# Autodesk Inventor assembly: stresstestingassembly
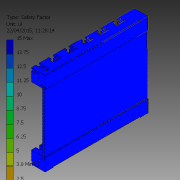
[picture p0: Inventor's stored thumbnail of the model, 180x180]
Saved by Autodesk Inventor 2015 (Build 190159000, 159)
## iProperties
Created: 2015-04-22
Part Number: stresstestingassembly
Document SubType Name: Assembly
Designer: Akovo_000
Author: Akovo_000
## Documents named in this file (9)
- C:\Users\Akovo_000\SkyDrive\3D printing\Enclosure Half-Open\stresstestingassembly.iam
- C:\Users\Akovo_000\SkyDrive\3D printing\Enclosure Half-Open\Pillar.ipt
- C:\Users\Akovo_000\SkyDrive\3D printing\Enclosure Half-Open\SidePanelNarrow.ipt
- C:\Users\Akovo_000\SkyDrive\3D printing\Enclosure Half-Open\stresstestingassembly\AIP\FEA\be9qf395s.fins
- C:\Users\Akovo_000\SkyDrive\3D printing\Enclosure Half-Open\stresstestingassembly\AIP\FEA\be9qf395s.fsat
- C:\Users\Akovo_000\SkyDrive\3D printing\Enclosure Half-Open\stresstestingassembly\AIP\FEA\be9qf396o.ftes
- C:\Users\Akovo_000\SkyDrive\3D printing\Enclosure Half-Open\stresstestingassembly\AIP\FEA\be9qf396o.fwiz
- C:\Users\Akovo_000\SkyDrive\3D printing\Enclosure Half-Open\stresstestingassembly\AIP\FEA\be9qf398g.fmsh
- C:\Users\Akovo_000\SkyDrive\3D printing\Enclosure Half-Open\stresstestingassembly\AIP\FEA\be9qf398h.fres
## Components (3 placed, 2 different names)
1. Pillar:1 — Slider:1
2. Pillar:3 — Slider:2
3. SidePanelNarrow:1 — Slider:1, Slider:2
## Relationships (2: TranslationJoint 2)
- Slider:1 [TranslationJoint]: Pillar:1 ↔ SidePanelNarrow:1
- Slider:2 [TranslationJoint]: Pillar:3 ↔ SidePanelNarrow:1
## Named parameters: sa_0 = 5000
note: some values were not read from the file. Shown as the stored number, unit unknown: "sa_0".
